# Autodesk Inventor assembly: Motor and Wheel
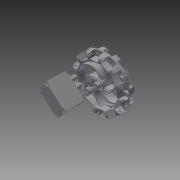
[picture p0: Inventor's stored thumbnail of the model, 180x180]
Saved by Autodesk Inventor 2015 (Build 190159000, 159)
## iProperties
Created: 2016-09-21
Part Number: Motor and Wheel
Document SubType Name: Assembly
Designer: Leo
Author: Leo
## Documents named in this file (5)
- C:\Users\Leo\Google Drive\StarStuckProject\Starstruck\Prototypes\Motor and Wheel.iam
- C:\Users\Leo\Google Drive\StarStuckProject\Starstruck\VEX Parts\Motion\Wheels\4in Omni Wheel Casing.iam
- C:\Users\Leo\Google Drive\StarStuckProject\Starstruck\Imported Components\Axle 4in\Axle 4in.ipt
- C:\Users\Leo\Google Drive\StarStuckProject\Starstruck\VEX Parts\Electronics\Compulsory\393 Motor Casing.iam
- C:\Users\Leo\Google Drive\StarStuckProject\Starstruck\Imported Components\Shaft Collar\Shaft Collar.ipt
## Components (6 placed, 4 different names)
1. 4in Omni Wheel Casing:1 [sub-assembly] — Mate:6, Mate:7
2. Axle 4in:1 — Tangent:5, Tangent:6, Tangent:7, Tangent:8, Tangent:9, Tangent:10
3. 393 Motor Casing:1 [sub-assembly]
4. Shaft Collar:1 — Tangent:5, Tangent:6, Mate:7
5. Shaft Collar:2 — Tangent:9, Tangent:10, Mate:6
6. Shaft Collar:3 — Tangent:7, Tangent:8
## Relationships (13: Mate 7, Tangent 6)
- [Mate]: 4in Omni Wheel Casing:1 ↔ Axle 4in:1
- [Mate]: 4in Omni Wheel Casing:1 ↔ Axle 4in:1
- [Mate]: Axle 4in:1 ↔ 393 Motor Casing:1
- [Mate]: Axle 4in:1 ↔ 393 Motor Casing:1
- [Mate]: Axle 4in:1 ↔ 393 Motor Casing:1
- Tangent:5 (-3.7338 mm): Axle 4in:1 ↔ Shaft Collar:1
- Tangent:6 (-3.7338 mm): Axle 4in:1 ↔ Shaft Collar:1
- Tangent:7 (-3.7338 mm): Axle 4in:1 ↔ Shaft Collar:3
- Tangent:8 (-3.7338 mm): Axle 4in:1 ↔ Shaft Collar:3
- Tangent:9 (-3.7338 mm): Axle 4in:1 ↔ Shaft Collar:2
- Tangent:10 (-3.7338 mm): Axle 4in:1 ↔ Shaft Collar:2
- Mate:6: 4in Omni Wheel Casing:1 ↔ Shaft Collar:2
- Mate:7: 4in Omni Wheel Casing:1 ↔ Shaft Collar:1
## Named parameters: d34_d30 = 0 mm, d35_d31 = 0 mm, d36_d32 = 0 mm, d37_d33 = 0 mm, d38_d29 = 0 mm
